# Autodesk Inventor assembly: Цилиндрическое зубчатое зацепление
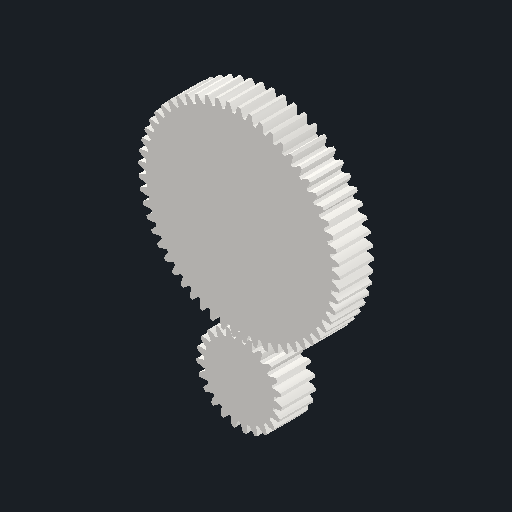
[picture p0: Inventor's stored thumbnail of the model, 512x512]
Saved by Autodesk Inventor 2025 (Build 290162000, 162)
## iProperties
ClientObjectVersion: 1
Created: 2025-01-15
Part Number: Цилиндрическое зубчатое зацепление
Document SubType Name: Assembly
Designer: Phantom
Categories: <?xml version="1.0" encoding="UTF-16"?> <MemberInstance><Categories><FamilyTemplate/><ParamToTemplateMap><ParamToTemplate><ParamToTemplate CategoryParameter="//CategoryParameter[@InternalName='9E91F9C2-1A37-4abf-91CE-B4CF7EE75BC6']" ConstantValue="10000000.000000"/></ParamToTemplate><ParamToTemplate><ParamToTemplate CategoryParameter="//CategoryParameter[@InternalName='2AFF4D85-1BD8-4ea8-8D18-96A2CAB0895B']" ConstantValue="9800000.000000"/></ParamToTemplate><ParamToTemplate><ParamToTemplate CategoryParameter="//CategoryParameter[@InternalName='E8E51088-10FD-40b5-B945-790B32C7EFBA']" ConstantValue="104.719755"/></ParamToTemplate><ParamToTemplate><ParamToTemplate CategoryParameter="//CategoryParameter[@InternalName='752D88A1-A866-440c-81C2-59259440B19C']" ConstantValue="42.255340"/></ParamToTemplate><ParamToTemplate><ParamToTemplate CategoryParameter="//CategoryParameter[@InternalName='5F43FD89-24D7-49f6-B63B-C3D8E39D8A69']" ConstantValue="95492.965855"/></ParamToTemplate><ParamToTemplate><ParamToTemplate CategoryParameter="//CategoryParameter[@InternalName='8D239626-6A17-497c-A9EF-C1C80B41D68F']" ConstantValue="231923.350986"/></ParamToTemplate><ParamToTemplate><ParamToTemplate CategoryParameter="//CategoryParameter[@InternalName='41D48E04-51D6-4192-AEE3-C42B8672B6EA']" ConstantValue="0.980000"/></ParamToTemplate><ParamToTemplate><ParamToTemplate CategoryParameter="//CategoryParameter[@InternalName='E5FFB0D5-AABD-4279-8B19-7DCFF75B68C0']" ConstantValue="6"/></ParamToTemplate></ParamToTemplateMap><Category DisplayName="Gears" InternalName="3565AA18-AB10-415a-941E-C703DB507537" Mnemonic="Gears"><CategoryParameter DisplayName="P" InternalName="9E91F9C2-1A37-4abf-91CE-B4CF7EE75BC6" Mnemonic="P1"/><CategoryParameter DisplayName="P" InternalName="2AFF4D85-1BD8-4ea8-8D18-96A2CAB0895B" Mnemonic="P2"/><CategoryParameter DisplayName="n" InternalName="E8E51088-10FD-40b5-B945-790B32C7EFBA" Mnemonic="n1"/><CategoryParameter DisplayName="n" InternalName="752D88A1-A866-440c-81C2-59259440B19C" Mnemonic="n2"/><CategoryParameter DisplayName="T" InternalName="5F43FD89-24D7-49f6-B63B-C3D8E39D8A69" Mnemonic="Mk1"/><CategoryParameter DisplayName="T" InternalName="8D239626-6A17-497c-A9EF-C1C80B41D68F" Mnemonic="Mk2"/><CategoryParameter DisplayName="||h|" InternalName="41D48E04-51D6-4192-AEE3-C42B8672B6EA" Mnemonic="eta"/><Category DisplayName="SpurGears" InternalName="B2B51C2B-6DC6-4009-A81E-78A8221B7E56" Mnemonic="SpurGears"><CategoryParameter DisplayName="idxIT1" InternalName="E5FFB0D5-AABD-4279-8B19-7DCFF75B68C0" Mnemonic="idxIT1"/></Category></Category></Categories></MemberInstance>
Author: Phantom
## Documents named in this file (3)
- C:\Users\Phantom\Desktop\Phantom16950\манипулятор шестерни\Мастер проектирования\Цилиндрическое зубчатое зацепление1.iam
- C:\Users\Phantom\Desktop\Phantom16950\манипулятор шестерни\Мастер проектирования\Цилиндрическое зубчатое зацепление11.ipt
- C:\Users\Phantom\Desktop\Phantom16950\манипулятор шестерни\Мастер проектирования\Цилиндрическое зубчатое зацепление21.ipt
## Components (2 placed, 2 different names)
1. Цилиндрическое зубчатое зацепление1:1 — Заподлицо:1, Совмещение:1, ЗубчПер:1
2. Цилиндрическое зубчатое зацепление2:1 — Заподлицо:1, Совмещение:1, ЗубчПер:1
## Relationships (3: Flush 1, Mate 1, RelateRotation 1)
- Заподлицо:1 [Flush]: Цилиндрическое зубчатое зацепление1:1 ↔ Цилиндрическое зубчатое зацепление2:1
- Совмещение:1 [Mate] (80 mm): Цилиндрическое зубчатое зацепление1:1 ↔ Цилиндрическое зубчатое зацепление2:1
- ЗубчПер:1 [RelateRotation] (0.4035 ul): Цилиндрическое зубчатое зацепление1:1 ↔ Цилиндрическое зубчатое зацепление2:1
